# Autodesk Inventor assembly: Unit_MR-I
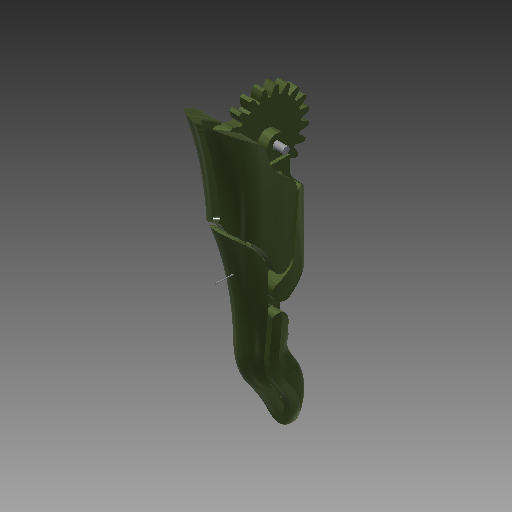
[picture p0: Inventor's stored thumbnail of the model, 512x512]
Saved by Autodesk Inventor 2018.2 (Build 222227000, 227)
## iProperties
Created: 2017-09-22
Part Number: Unit_MR-I
Material: 一般
Document SubType Name: Assembly
Designer: sktom
Author: sktom
Title: Unit_MR-I
## Documents named in this file (12)
- D:\CloudStrage\OneDrive\CADMech\HbSizeMMech\UnitHand\Unit_MR-H\Unit_MR-I\Unit_MR-I .iam
- D:\CloudStrage\OneDrive\CADMech\HbSizeMMech\UnitHand\Unit_MR-H\Unit_MR-I\Dummy_Position.ipt
- D:\CloudStrage\OneDrive\CADMech\HbSizeMMech\UnitHand\Unit_MR-H\Unit_MR-I\MR-I-01.ipt
- D:\CloudStrage\OneDrive\CADMech\HbSizeMMech\UnitHand\Unit_MR-H\Unit_MR-I\MR-I-02.ipt
- D:\CloudStrage\OneDrive\CADMech\HbSizeMMech\UnitHand\Unit_MR-H\Unit_MR-I\MR-I-04.ipt
- D:\CloudStrage\OneDrive\CADMech\HbSizeMMech\UnitHand\Unit_MR-H\Unit_MR-I\MR-I-05.ipt
- D:\CloudStrage\OneDrive\CADMech\HbSizeMMech\UnitHand\Unit_MR-H\Unit_MR-I\MR-I-06.ipt
- D:\CloudStrage\OneDrive\CADMech\HbSizeMMech\UnitHand\Unit_MR-H\Unit_MR-I\MR-I-07.ipt
- D:\CloudStrage\OneDrive\CADMech\HbSizeMMech\UnitHand\Unit_MR-H\Unit_MR-I\Parts_Screw_M1.7_L8.ipt
- D:\CloudStrage\OneDrive\CADMech\HbSizeMMech\UnitHand\Unit_MR-H\Unit_MR-I\MR-I-03.ipt
- D:\CloudStrage\OneDrive\CADMech\HbSizeMMech\UnitHand\Unit_MR-H\Unit_MR-I\Parts_Shaft_Phi2_L8.ipt
- D:\CloudStrage\OneDrive\CADMech\HbSizeMMech\UnitHand\Unit_MR-H\Unit_MR-I\Parts_TorsionSpring_TOS 0.3-4-270ﾟ-3.ipt
## Components (16 placed, 11 different names)
1. Dummy_Position — 円柱状:1, 円柱状:2, 回転:1, 回転:2, 円柱状:4, 回転:3, 回転:4
2. MR-I-01 — 円柱状:1, 円柱状:2, メイト:1, 円柱状:3, 円柱状:5, メイト:2, メイト:3
3. MR-I-02 — 挿入:1, 挿入:2, 挿入:5, 挿入:6, 円柱状:3, 円柱状:4, メイト:2
4. MR-I-03 — 回転:2, 円柱状:6
5. MR-I-04 — 挿入:1, 挿入:2
6. MR-I-05 — 円柱状:7, メイト:4, 回転:5
7. MR-I-06 — 挿入:3, 挿入:4, 挿入:7, 挿入:8, 円柱状:5, 円柱状:6, メイト:3, 円柱状:7, メイト:4
8. MR-I-07 — 挿入:3, 挿入:4
9. Parts_Screw_M1.7_L8:1 — 挿入:8
10. Parts_Screw_M1.7_L8:2 — 挿入:7
11. Parts_Screw_M1.7_L8:3 — 挿入:5
12. Parts_Screw_M1.7_L8:4 — 挿入:6
13. Parts_Shaft_Phi2_L8:1 — 回転:4
14. Parts_Shaft_Phi2_L8:2 — 回転:3
15. Parts_Shaft_Phi2_L8:3 — 回転:5
16. Parts_TorsionSpring_TOS 0.3-4-270ﾟ-3:1 — 回転:1, メイト:1
## Relationships (24: Insert 8, CylindricalJoint 7, RevoluteJoint 5, Mate 4)
- 挿入:1 [Insert]: MR-I-02 ↔ MR-I-04
- 挿入:2 [Insert]: MR-I-02 ↔ MR-I-04
- 挿入:3 [Insert]: MR-I-06 ↔ MR-I-07
- 挿入:4 [Insert]: MR-I-06 ↔ MR-I-07
- 挿入:5 [Insert]: MR-I-02 ↔ Parts_Screw_M1.7_L8:3
- 挿入:6 [Insert]: MR-I-02 ↔ Parts_Screw_M1.7_L8:4
- 挿入:7 [Insert]: MR-I-06 ↔ Parts_Screw_M1.7_L8:2
- 挿入:8 [Insert]: MR-I-06 ↔ Parts_Screw_M1.7_L8:1
- 円柱状:1 [CylindricalJoint]: Dummy_Position ↔ MR-I-01
- 円柱状:2 [CylindricalJoint]: Dummy_Position ↔ MR-I-01
- 回転:1 [RevoluteJoint]: Dummy_Position ↔ Parts_TorsionSpring_TOS 0.3-4-270ﾟ-3:1
- メイト:1 [Mate] (0.028 mm): MR-I-01 ↔ Parts_TorsionSpring_TOS 0.3-4-270ﾟ-3:1
- 回転:2 [RevoluteJoint]: Dummy_Position ↔ MR-I-03
- 円柱状:3 [CylindricalJoint]: MR-I-01 ↔ MR-I-02
- 円柱状:4 [CylindricalJoint]: Dummy_Position ↔ MR-I-02
- 円柱状:5 [CylindricalJoint]: MR-I-01 ↔ MR-I-06
- メイト:2 [Mate] (0.44 mm): MR-I-01 ↔ MR-I-02
- 円柱状:6 [CylindricalJoint]: MR-I-03 ↔ MR-I-06
- メイト:3 [Mate] (0.35 mm): MR-I-01 ↔ MR-I-06
- 円柱状:7 [CylindricalJoint]: MR-I-05 ↔ MR-I-06
- メイト:4 [Mate] (0.49 mm): MR-I-05 ↔ MR-I-06
- 回転:3 [RevoluteJoint]: Dummy_Position ↔ Parts_Shaft_Phi2_L8:2
- 回転:4 [RevoluteJoint]: Dummy_Position ↔ Parts_Shaft_Phi2_L8:1
- 回転:5 [RevoluteJoint]: MR-I-05 ↔ Parts_Shaft_Phi2_L8:3
